# Autodesk Inventor assembly: Ensamblaje2
(part 3 of 3)
- Insertar:648: Tornillo Allen cabeza botón M4x20mm:38 ↔ Arandela Plana Tipo A DIN 125 - M4:13
- Insertar:649: Tornillo Allen cabeza botón M4x20mm:39 ↔ Arandela Plana Tipo A DIN 125 - M4:14
- Insertar:650: Tornillo Allen cabeza botón M4x20mm:40 ↔ Arandela Plana Tipo A DIN 125 - M4:15
- Insertar:651: Tornillo Allen cabeza botón M4x20mm:41 ↔ Arandela Plana Tipo A DIN 125 - M4:16
- Insertar:652: Tornillo Allen cabeza botón M4x20mm:42 ↔ Arandela Plana Tipo A DIN 125 - M4:17
- Insertar:653: Techo Carcasa:1 ↔ Arandela Plana Tipo A DIN 125 - M4:14
- Insertar:654: Techo Carcasa:1 ↔ Arandela Plana Tipo A DIN 125 - M4:15
- Insertar:655: Lateral Izquierdo Carcasa:1 ↔ Arandela Plana Tipo A DIN 125 - M4:16
- Insertar:656: Lateral Izquierdo Carcasa:1 ↔ Arandela Plana Tipo A DIN 125 - M4:17
- Insertar:657: Lateral Izquierdo Carcasa:1 ↔ Arandela Plana Tipo A DIN 125 - M4:6
- Insertar:658: Culata Carcaza:1 ↔ Arandela Plana Tipo A DIN 125 - M4:7
- Insertar:659: Culata Carcaza:1 ↔ Arandela Plana Tipo A DIN 125 - M4:8
- Insertar:660: Lateral Izquierdo Carcasa:1 ↔ Arandela Plana Tipo A DIN 125 - M4:9
- Insertar:661: Lateral Izquierdo Carcasa:1 ↔ Arandela Plana Tipo A DIN 125 - M4:10
- Insertar:662: Culata Carcaza:1 ↔ Arandela Plana Tipo A DIN 125 - M4:11
- Insertar:663: Culata Carcaza:1 ↔ Arandela Plana Tipo A DIN 125 - M4:12
- Insertar:664: Lateral Izquierdo Carcasa:1 ↔ Arandela Plana Tipo A DIN 125 - M4:13
- Insertar:665: Lateral Derecho Carcasa:1 ↔ Arandela Plana Tipo A DIN 125 - M4:34
- Insertar:666: Lateral Izquierdo Carcasa:1 ↔ Arandela Plana Tipo A DIN 125 - M4:35
- Coincidencia:404 [Mate]: Cielo raso:1 ↔ ISO 4032 M6:1
- Insertar:667: Cielo raso:1 ↔ ISO 4032 M6:2
- Insertar:668: Cielo raso:1 ↔ ISO 4032 M6:3
- Insertar:669: Cielo raso:1 ↔ ISO 4032 M6:4
- Insertar:670: Cielo raso:1 ↔ ISO 4032 M6:5
- Insertar:671: Cielo raso:1 ↔ ISO 4032 M6:8
- Insertar:672: Cielo raso:1 ↔ ISO 4032 M6:6
- Insertar:673: Cielo raso:1 ↔ ISO 4032 M6:9
- Insertar:674: Cielo raso:1 ↔ ISO 4032 M6:10
- Insertar:675: Cielo raso:1 ↔ ISO 4032 M6:11
- Coincidencia:405 [Mate]: Tornillo Allen cabeza botón M4x20mm:23 ↔ ISO 4032 M4:1
- Coincidencia:406 [Mate]: Chapa Base:1 ↔ ISO 4032 M4:1
- Insertar:676: Chapa Base:1 ↔ ISO 4032 M4:2
- Insertar:677: Tornillo Allen cabeza botón M6x16mm:20 ↔ Arandela plana tipo A DIN 125 M6:34
- Insertar:678: Tornillo Allen cabeza botón M6x16mm:21 ↔ Arandela plana tipo A DIN 125 M6:35
- Insertar:679: Tornillo Allen cabeza botón M6x16mm:22 ↔ Arandela plana tipo A DIN 125 M6:36
- Insertar:680: Tornillo Allen cabeza botón M6x16mm:23 ↔ Arandela plana tipo A DIN 125 M6:37
- Insertar:681: Tornillo Allen cabeza botón M6x16mm:24 ↔ Arandela plana tipo A DIN 125 M6:41
- Insertar:682: Tornillo Allen cabeza botón M6x16mm:25 ↔ Arandela plana tipo A DIN 125 M6:42
- Insertar:683: Tornillo Allen cabeza botón M6x16mm:26 ↔ Arandela plana tipo A DIN 125 M6:43
- Insertar:684: Tornillo Allen cabeza botón M6x16mm:27 ↔ Arandela plana tipo A DIN 125 M6:38
- Insertar:685: Tornillo Allen cabeza botón M6x16mm:28 ↔ Arandela plana tipo A DIN 125 M6:39
- Insertar:686: Tornillo Allen cabeza botón M6x16mm:29 ↔ Arandela plana tipo A DIN 125 M6:40
- Insertar:687: Tornillo Allen cabeza botón M6x16mm:30 ↔ Arandela plana tipo A DIN 125 M6:44
- Insertar:688: Tornillo Allen cabeza botón M6x16mm:31 ↔ Arandela plana tipo A DIN 125 M6:45
- Insertar:689: Tornillo Allen cabeza botón M6x16mm:32 ↔ Arandela plana tipo A DIN 125 M6:46
- Insertar:690: Lateral Izquierdo Carcasa:1 ↔ Arandela plana tipo A DIN 125 M6:34
- Insertar:691: Lateral Izquierdo Carcasa:1 ↔ Arandela plana tipo A DIN 125 M6:35
- Insertar:692: Lateral Izquierdo Carcasa:1 ↔ Arandela plana tipo A DIN 125 M6:36
- Insertar:693: Frente Carcasa:1 ↔ Arandela plana tipo A DIN 125 M6:37
- Insertar:694: Frente Carcasa:1 ↔ Arandela plana tipo A DIN 125 M6:41
- Insertar:695: Frente Carcasa:1 ↔ Arandela plana tipo A DIN 125 M6:42
- Insertar:696: Frente Carcasa:1 ↔ Arandela plana tipo A DIN 125 M6:43
- Insertar:697: Frente Carcasa:1 ↔ Arandela plana tipo A DIN 125 M6:40
- Insertar:698: Frente Carcasa:1 ↔ Arandela plana tipo A DIN 125 M6:46
- Insertar:699: Frente Carcasa:1 ↔ Arandela plana tipo A DIN 125 M6:39
- Insertar:700: Lateral Derecho Carcasa:1 ↔ Arandela plana tipo A DIN 125 M6:38
- Insertar:701: Lateral Derecho Carcasa:1 ↔ Arandela plana tipo A DIN 125 M6:45
- Insertar:702: Lateral Derecho Carcasa:1 ↔ Arandela plana tipo A DIN 125 M6:44
- Insertar:703: Arandela plana tipo A DIN 125 M6:16 ↔ Tornillo Allen cabeza botón M6x16mm:33
- Insertar:704: Arandela plana tipo A DIN 125 M6:17 ↔ Tornillo Allen cabeza botón M6x16mm:34
- Insertar:705: Arandela plana tipo A DIN 125 M6:18 ↔ Tornillo Allen cabeza botón M6x16mm:35
- Insertar:706: Arandela plana tipo A DIN 125 M6:28 ↔ Tornillo Allen cabeza botón M6x16mm:36
- Insertar:707: Arandela plana tipo A DIN 125 M6:29 ↔ Tornillo Allen cabeza botón M6x16mm:37
- Insertar:708: Arandela plana tipo A DIN 125 M6:30 ↔ Tornillo Allen cabeza botón M6x16mm:38
- Insertar:715: Lateral Izquierdo Carcasa:1 ↔ Arandela plana tipo A DIN 125-M5:1
- Insertar:716: Lateral Izquierdo Carcasa:1 ↔ Arandela plana tipo A DIN 125-M5:2
- Insertar:717: Lateral Izquierdo Carcasa:1 ↔ Arandela plana tipo A DIN 125-M5:3
- Insertar:718: Lateral Izquierdo Carcasa:1 ↔ Arandela plana tipo A DIN 125-M5:6
- Insertar:719: Lateral Izquierdo Carcasa:1 ↔ Arandela plana tipo A DIN 125-M5:5
- Insertar:720: Lateral Izquierdo Carcasa:1 ↔ Arandela plana tipo A DIN 125-M5:4
- Insertar:721: Arandela plana tipo A DIN 125-M5:1 ↔ ISO 4032 M5:3
- Insertar:722: Ala 1 Bisagra tipo T:1 ↔ Tornillo allen cabeza boton M5x16mm:3
- Insertar:723: Ala 1 Bisagra tipo T:1 ↔ Tornillo allen cabeza boton M5x16mm:1
- Insertar:724: Ala 1 Bisagra tipo T:1 ↔ Tornillo allen cabeza boton M5x16mm:2
- Insertar:725: Ala 1 Bisagra tipo T:2 ↔ Tornillo allen cabeza boton M5x16mm:4
- Insertar:726: Ala 1 Bisagra tipo T:2 ↔ Tornillo allen cabeza boton M5x16mm:5
- Insertar:727: Ala 1 Bisagra tipo T:2 ↔ Tornillo allen cabeza boton M5x16mm:6
- Insertar:728: Arandela plana tipo A DIN 125-M5:2 ↔ ISO 4032 M5:1
- Insertar:729: Arandela plana tipo A DIN 125-M5:3 ↔ ISO 4032 M5:2
- Insertar:730: Arandela plana tipo A DIN 125-M5:6 ↔ ISO 4032 M5:4
- Insertar:731: Arandela plana tipo A DIN 125-M5:5 ↔ ISO 4032 M5:5
- Insertar:732: Arandela plana tipo A DIN 125-M5:4 ↔ ISO 4032 M5:6
- Insertar:733: Chapon:1 ↔ Tornillo Allen cabeza botón M4x10mm:7
- Insertar:734: Chapon:1 ↔ Tornillo Allen cabeza botón M4x10mm:8
- Insertar:739: Tornillo Allen cabeza botón M4x20mm:47 ↔ Arandela Plana Tipo A DIN 125 - M4:42
- Insertar:740: Tornillo Allen cabeza botón M4x20mm:48 ↔ Arandela Plana Tipo A DIN 125 - M4:43
- Insertar:741: Tornillo Allen cabeza botón M4x20mm:49 ↔ Arandela Plana Tipo A DIN 125 - M4:44
- Insertar:742: Tornillo Allen cabeza botón M4x20mm:50 ↔ Arandela Plana Tipo A DIN 125 - M4:45
- Insertar:743: Culata Carcaza:1 ↔ Arandela Plana Tipo A DIN 125 - M4:42
- Insertar:744: Culata Carcaza:1 ↔ Arandela Plana Tipo A DIN 125 - M4:43
- Insertar:745: Culata Carcaza:1 ↔ Arandela Plana Tipo A DIN 125 - M4:44
- Insertar:746: Culata Carcaza:1 ↔ Arandela Plana Tipo A DIN 125 - M4:45
- Insertar:747: Travesaño Estructural:1 ↔ Tornillo Allen cabeza botón M4x20mm:43
- Insertar:748: Travesaño Estructural:1 ↔ Tornillo Allen cabeza botón M4x20mm:44
- Insertar:749: Travesaño Estructural:1 ↔ Tornillo Allen cabeza botón M4x20mm:46
- Insertar:750: Travesaño Estructural:1 ↔ Tornillo Allen cabeza botón M4x20mm:45
- Insertar:755: Ala 2 Bisagra tipo Libro Grande:2 ↔ Puerta Lateral Derecha:1
- Insertar:756: Ala 2 Bisagra tipo Libro Grande:1 ↔ Puerta Lateral Derecha:1
- Insertar:757: Ala 2 Bisagra tipo Libro Chica:2 ↔ Puerta de Inspección:1
- Coincidencia:407 [Mate]: Ala 2 Bisagra tipo Libro Chica:1 ↔ Puerta de Inspección:1
- Coincidencia:408 [Mate]: Ala 2 Bisagra tipo Libro Chica:1 ↔ Puerta de Inspección:1
- Insertar:764: Ala 2 Bisagra tipo Libro Chica:2 ↔ Tornillo Allen cabeza botón M4x10mm:15
- Insertar:765: Ala 2 Bisagra tipo Libro Chica:2 ↔ Tornillo Allen cabeza botón M4x10mm:16
- Insertar:766: Ala 2 Bisagra tipo Libro Chica:2 ↔ Tornillo Allen cabeza botón M4x10mm:17
- Insertar:767: Ala 2 Bisagra tipo Libro Chica:1 ↔ Tornillo Allen cabeza botón M4x10mm:20
- Insertar:768: Ala 2 Bisagra tipo Libro Chica:1 ↔ Tornillo Allen cabeza botón M4x10mm:19
- Insertar:769: Ala 2 Bisagra tipo Libro Chica:1 ↔ Tornillo Allen cabeza botón M4x10mm:18
- Insertar:772: Ala 2 Bisagra tipo Libro Grande:1 ↔ Tornillo Allen cabeza botón M4x10mm:23
- Insertar:773: Ala 2 Bisagra tipo Libro Grande:1 ↔ Tornillo Allen cabeza botón M4x10mm:24
- Insertar:774: Ala 2 Bisagra tipo Libro Grande:1 ↔ Tornillo Allen cabeza botón M4x10mm:28
- Insertar:775: Ala 2 Bisagra tipo Libro Grande:2 ↔ Tornillo Allen cabeza botón M4x10mm:25
- Insertar:776: Ala 2 Bisagra tipo Libro Grande:2 ↔ Tornillo Allen cabeza botón M4x10mm:27
- Insertar:777: Ala 2 Bisagra tipo Libro Grande:2 ↔ Tornillo Allen cabeza botón M4x10mm:26
- Insertar:780: Lateral Derecho Carcasa:1 ↔ Arandela Plana Tipo A DIN 125 - M4:49
- Insertar:781: Lateral Derecho Carcasa:1 ↔ Arandela Plana Tipo A DIN 125 - M4:47
- Insertar:782: Lateral Derecho Carcasa:1 ↔ Arandela Plana Tipo A DIN 125 - M4:46
- Insertar:783: Lateral Derecho Carcasa:1 ↔ Arandela Plana Tipo A DIN 125 - M4:52
- Insertar:784: Techo Carcasa:1 ↔ Arandela Plana Tipo A DIN 125 - M4:50
- Insertar:785: Techo Carcasa:1 ↔ Arandela Plana Tipo A DIN 125 - M4:51
- Insertar:786: Techo Carcasa:1 ↔ Arandela Plana Tipo A DIN 125 - M4:53
- Insertar:787: Techo Carcasa:1 ↔ Arandela Plana Tipo A DIN 125 - M4:54
- Insertar:788: Techo Carcasa:1 ↔ Arandela Plana Tipo A DIN 125 - M4:55
- Insertar:789: Techo Carcasa:1 ↔ Arandela Plana Tipo A DIN 125 - M4:48
- Insertar:790: ISO 4032 M4:3 ↔ Arandela Plana Tipo A DIN 125 - M4:50
- Insertar:791: ISO 4032 M4:4 ↔ Arandela Plana Tipo A DIN 125 - M4:51
- Insertar:792: ISO 4032 M4:5 ↔ Arandela Plana Tipo A DIN 125 - M4:53
- Insertar:793: ISO 4032 M4:6 ↔ Arandela Plana Tipo A DIN 125 - M4:54
- Insertar:794: ISO 4032 M4:7 ↔ Arandela Plana Tipo A DIN 125 - M4:55
- Insertar:795: ISO 4032 M4:8 ↔ Arandela Plana Tipo A DIN 125 - M4:48
- Insertar:796: ISO 4032 M4:9 ↔ Arandela Plana Tipo A DIN 125 - M4:52
- Insertar:797: ISO 4032 M4:10 ↔ Arandela Plana Tipo A DIN 125 - M4:46
- Insertar:798: ISO 4032 M4:11 ↔ Arandela Plana Tipo A DIN 125 - M4:49
- Insertar:799: ISO 4032 M4:12 ↔ Arandela Plana Tipo A DIN 125 - M4:47
- Insertar:800: Puerta de Inspección:1 ↔ ISO 4032 M4:13
- Insertar:801: Puerta de Inspección:1 ↔ ISO 4032 M4:14
- Insertar:802: Puerta de Inspección:1 ↔ ISO 4032 M4:15
- Insertar:803: Puerta de Inspección:1 ↔ ISO 4032 M4:16
- Insertar:804: Puerta de Inspección:1 ↔ ISO 4032 M4:17
- Insertar:805: Puerta de Inspección:1 ↔ ISO 4032 M4:18
- Insertar:806: Puerta Lateral Derecha:1 ↔ ISO 4032 M4:19
- Insertar:807: Puerta Lateral Derecha:1 ↔ ISO 4032 M4:20
- Insertar:808: Puerta Lateral Derecha:1 ↔ ISO 4032 M4:21
- Insertar:809: Puerta Lateral Derecha:1 ↔ ISO 4032 M4:22
- Insertar:810: Puerta Lateral Derecha:1 ↔ ISO 4032 M4:23
- Insertar:811: Puerta Lateral Derecha:1 ↔ ISO 4032 M4:24
- Insertar:812: Ala 2 Bisagra tipo T:1 ↔ Tornillo allen cabeza boton M5x10mm:1
- Insertar:813: Ala 2 Bisagra tipo T:1 ↔ Tornillo allen cabeza boton M5x10mm:2
- Insertar:814: Ala 2 Bisagra tipo T:2 ↔ Tornillo allen cabeza boton M5x10mm:3
- Insertar:815: Ala 2 Bisagra tipo T:2 ↔ Tornillo allen cabeza boton M5x10mm:4
- Ángulo:4 [Angle] (0 deg): Lateral Izquierdo Carcasa:1 ↔ Puerta de Inspección:1
- Insertar:816: Chapon:1 ↔ Soporte para culata carcasa:2
- Insertar:817: Chapon:1 ↔ Soporte para culata carcasa:1
- Insertar:818: Chapon:1 ↔ Soporte para culata carcasa:1
- Insertar:819: Chapon:1 ↔ Soporte para culata carcasa:2
- Coincidencia:409 [Mate]: Ala 2 Bisagra tipo T:1 ↔ Puerta Frontal:1
- Coincidencia:410 [Mate]: Ala 2 Bisagra tipo T:2 ↔ Puerta Frontal:1
- Insertar:826: Ala 2 Bisagra tipo T:1 ↔ Puerta Frontal:1
- Insertar:827: Ala 2 Bisagra tipo T:2 ↔ Puerta Frontal:1
- Insertar:828: Cielo raso:1 ↔ Tornillo Allen cabeza botón M4x10mm:56
- Insertar:829: Cielo raso:1 ↔ Tornillo Allen cabeza botón M4x10mm:55
- Insertar:830: Chapon:1 ↔ ISO 4032 M4:25
- Insertar:831: Chapon:1 ↔ ISO 4032 M4:26
- Insertar:832: Ala 1 Bisagra tipo Libro Grande:1 ↔ Tornillo Allen cabeza botón M4x16mm:7
- Insertar:833: Ala 1 Bisagra tipo Libro Grande:1 ↔ Tornillo Allen cabeza botón M4x16mm:8
- Insertar:834: Ala 1 Bisagra tipo Libro Grande:2 ↔ Tornillo Allen cabeza botón M4x16mm:9
- Insertar:835: Ala 1 Bisagra tipo Libro Grande:2 ↔ Tornillo Allen cabeza botón M4x16mm:10
- Insertar:836: Ala 1 Bisagra tipo Libro Chica:1 ↔ Tornillo Allen cabeza botón M4x16mm:5
- Insertar:837: Ala 1 Bisagra tipo Libro Chica:1 ↔ Tornillo Allen cabeza botón M4x16mm:4
- Insertar:838: Ala 1 Bisagra tipo Libro Chica:1 ↔ Tornillo Allen cabeza botón M4x16mm:3
- Insertar:839: Ala 1 Bisagra tipo Libro Chica:2 ↔ Tornillo Allen cabeza botón M4x16mm:2
- Insertar:840: Ala 1 Bisagra tipo Libro Chica:2 ↔ Tornillo Allen cabeza botón M4x16mm:1
- Insertar:841: Ala 1 Bisagra tipo Libro Chica:2 ↔ Tornillo Allen cabeza botón M4x16mm:6
- Insertar:842: Puerta Frontal:1 ↔ ISO 4032 M4:27
- Insertar:843: Puerta Frontal:1 ↔ ISO 4032 M4:28
- Insertar:844: Puerta Frontal:1 ↔ ISO 4032 M4:29
- Insertar:845: Puerta Frontal:1 ↔ ISO 4032 M4:30
- Insertar:846: Soporte de Final de Carrera - Eje Y:1 ↔ Tornillo Allen cabeeza botón M3x8mm:33
- Insertar:847: Soporte de Final de Carrera - Eje Y:1 ↔ Tornillo Allen cabeeza botón M3x8mm:34
- Coincidencia:411 [Mate]: Tornillo Allen cabeza cilindrica M2x16mm:7 ↔ ISO 4032 M2:1
- Coincidencia:412 [Mate]: Soporte de Final de Carrera - Eje Y:1 ↔ ISO 4032 M2:1
- Coincidencia:413 [Mate]: Tornillo Allen cabeza cilindrica M2x16mm:6 ↔ ISO 4032 M2:2
- Coincidencia:414 [Mate]: Soporte de Final de Carrera - Eje Y:1 ↔ ISO 4032 M2:2
- Coincidencia:415 [Mate]: Tornillo Allen cabeeza botón M3x8mm:33 ↔ ISO 4032 M3:1
- Coincidencia:416 [Mate]: Chapon:1 ↔ ISO 4032 M3:1
- Coincidencia:417 [Mate]: Tornillo Allen cabeeza botón M3x8mm:34 ↔ ISO 4032 M3:2
- Coincidencia:418 [Mate]: Chapon:1 ↔ ISO 4032 M3:2
- Ángulo:7 [Angle] (0 deg): Frente Carcasa:1 ↔ Puerta Frontal:1
- Ángulo:8 [Angle] (0 deg): Lateral Derecho Carcasa:1 ↔ Puerta Lateral Derecha:1
- Coincidencia:419 [Mate]: Tornillo Allen cabeza cilindrica M2x16mm:3 ↔ ISO 4032 M2:3
- Coincidencia:420 [Mate]: Soporte de Final de Carrera - Eje X:1 ↔ ISO 4032 M2:3
- Coincidencia:421 [Mate]: Tornillo Allen cabeza cilindrica M2x16mm:4 ↔ ISO 4032 M2:4
- Coincidencia:422 [Mate]: Soporte de Final de Carrera - Eje X:1 ↔ ISO 4032 M2:4
- Insertar:852: Bloque - Vinculo Cabezal:1 ↔ Kit sugecion 1:1
- Insertar:853: Bloque - Vinculo Cabezal:1 ↔ Kit sugecion 1:1
- Insertar:854: Cielo raso:1 ↔ Kit de sujecion 2:2
- Insertar:855: Cielo raso:1 ↔ Kit de sujecion 2:2
- Coincidencia:423 [Mate]: Soporte de tuerca de mesa:1 ↔ Eslabon cadena portacable:1
- Nivelación:60 [Flush] (-2.293 mm): Soporte de tuerca de mesa:1 ↔ Eslabon cadena portacable:1
- Insert:856: Kit sugecion 1:1 ↔ Tornillo Allen cabeeza botón M3x8mm:35
- Insert:857: Kit sugecion 1:1 ↔ Tornillo Allen cabeeza botón M3x8mm:36
- Insert:858: Kit de sujecion 2:2 ↔ Tornillo Allen cabeeza botón M3x16mm:1
- Insert:859: Kit de sujecion 2:2 ↔ Tornillo Allen cabeeza botón M3x16mm:2
- Insert:860: Cielo raso:1 ↔ ISO 4032 M3:3
- Insert:861: Cielo raso:1 ↔ ISO 4032 M3:4
